# Autodesk Inventor assembly: Electromagnet
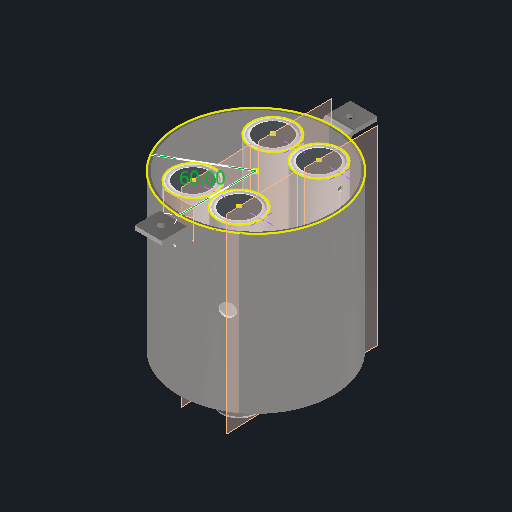
[picture p0: Inventor's stored thumbnail of the model, 512x512]
Saved by Autodesk Inventor 2026.3 (Build 303398000, 398)
## iProperties
Created: 2026-07-22
Part Number: Electromagnet
Document SubType Name: Assembly
Designer: matot
Author: matot
## Documents named in this file (5)
- C:\Users\matot\OneDrive - Stellenbosch University\2026\MechatronicsProject478\Building the joint\Joint Assembly\Electromagnet.iam
- C:\Users\matot\OneDrive - Stellenbosch University\2026\MechatronicsProject478\Building the joint\Joint Assembly\Solenoid core.ipt
- C:\Users\matot\OneDrive - Stellenbosch University\2026\MechatronicsProject478\Building the joint\Joint Assembly\Solenoid Yoke.ipt
- C:\Users\matot\OneDrive - Stellenbosch University\2026\MechatronicsProject478\Building the joint\Joint Assembly\Electromagnet cover.iam
- C:\Users\matot\OneDrive - Stellenbosch University\2026\MechatronicsProject478\Building the joint\Joint Assembly\Pressure plate tab_L.ipt
## Components (11 placed, 4 different names)
1. Solenoid core:1 — Insert:5
2. Solenoid core:2 — Insert:2
3. Solenoid core:3 — Insert:3
4. Solenoid core:4 — Insert:6
5. Solenoid Yoke:1 — Insert:2, Insert:12
6. Solenoid Yoke:2 — Insert:3, Insert:11
7. Solenoid Yoke:3 — Insert:5, Insert:9
8. Solenoid Yoke:4 — Insert:6, Insert:8
9. Electromagnet cover:1 [sub-assembly] — Insert:8, Insert:9, Insert:11, Insert:12, Tangent:1, Mate:1, Flush:1, Tangent:2, Mate:2, Flush:2
10. Pressure plate tab_L:1 — Tangent:1, Mate:1, Flush:1
11. Pressure plate tab_L:2 — Tangent:2, Mate:2, Flush:2
## Relationships (14: Insert 8, Tangent 2, Mate 2, Flush 2)
- Insert:2: Solenoid core:2 ↔ Solenoid Yoke:1
- Insert:3: Solenoid core:3 ↔ Solenoid Yoke:2
- Insert:5: Solenoid core:1 ↔ Solenoid Yoke:3
- Insert:6: Solenoid core:4 ↔ Solenoid Yoke:4
- Insert:8: Solenoid Yoke:4 ↔ Electromagnet cover:1
- Insert:9: Solenoid Yoke:3 ↔ Electromagnet cover:1
- Insert:11: Solenoid Yoke:2 ↔ Electromagnet cover:1
- Insert:12: Solenoid Yoke:1 ↔ Electromagnet cover:1
- Tangent:1: Electromagnet cover:1 ↔ Pressure plate tab_L:1
- Mate:1: Electromagnet cover:1 ↔ Pressure plate tab_L:1
- Flush:1: Electromagnet cover:1 ↔ Pressure plate tab_L:1
- Tangent:2: Electromagnet cover:1 ↔ Pressure plate tab_L:2
- Mate:2: Electromagnet cover:1 ↔ Pressure plate tab_L:2
- Flush:2: Electromagnet cover:1 ↔ Pressure plate tab_L:2
